# Autodesk Inventor assembly: Baugruppe1
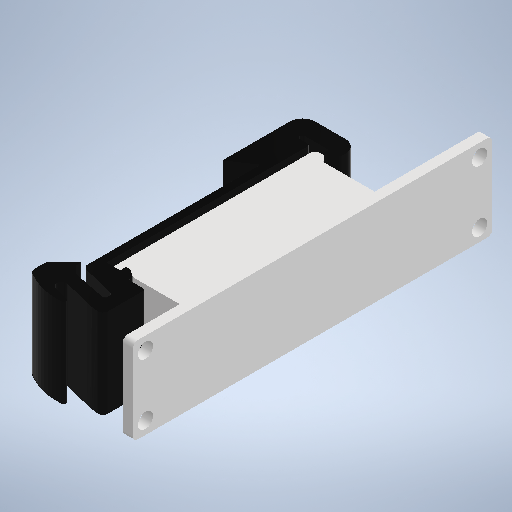
[picture p0: Inventor's stored thumbnail of the model, 512x512]
Saved by Autodesk Inventor 2025.2 (Build 292293000, 293)
## iProperties
Created: 2025-03-23
Part Number: Baugruppe1
Document SubType Name: Assembly
Designer: Quatana
Author: Quatana
## Documents named in this file (3)
- C:\Hauptspeicher\BZTG\ETS24\MC\005_Projekt_Kontrollpanel\Baugruppe1.iam
- C:\Hauptspeicher\BZTG\ETS24\MC\005_Projekt_Kontrollpanel\Relais_Platte.ipt
- C:\Users\Quatana\Downloads\SHWH_DIN_Klammer_V2.ipt
## Components (2 placed, 2 different names)
1. Relais_Platte:1 — Passend:1, Passend:2
2. SHWH_DIN_Klammer_V2:1 — Passend:1, Passend:2
## Relationships (2: Mate 2)
- Passend:1 [Mate]: Relais_Platte:1 ↔ SHWH_DIN_Klammer_V2:1
- Passend:2 [Mate]: Relais_Platte:1 ↔ SHWH_DIN_Klammer_V2:1
